# Autodesk Inventor assembly: 20220523_仮機体
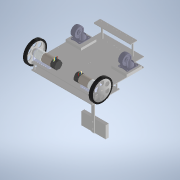
[picture p0: Inventor's stored thumbnail of the model, 180x180]
Saved by Autodesk Inventor 2020 (Build 240168000, 168)
## iProperties
Created: 2022-05-22
Part Number: 20220523_仮機体
Document SubType Name: Assembly
Designer: Naggy
Author: Naggy
## Documents named in this file (15)
- C:\Users\Naggy\Documents\Inventor\robot_design2020\20220523_仮機体.iam
- C:\Users\Naggy\Documents\Inventor\robot_design2020\20220522.ipt
- C:\Users\Naggy\Documents\Inventor\robot_design2020\20220509_知能ロボットキャスタ.ipt
- C:\Users\Naggy\Documents\Inventor\robot_design2020\20220519モータを取り付けるやつ.ipt
- C:\Users\Naggy\Documents\Inventor\robot_design2020\20220519知能ロボットモータとエンコーダ.ipt
- C:\Users\Naggy\Documents\Inventor\robot_design2020\70アルミホイール内径６ (1).ipt
- C:\Users\Naggy\Documents\Inventor\robot_design2020\RD003_キャスタ420G-R32 (3).ipt
- C:\Users\Naggy\Documents\Inventor\robot_design2020\20220508_知能ロボットスペーサ.ipt
- C:\Users\Naggy\Documents\Inventor\robot_design2020\20220523_知能ロボット2階部分.ipt
- C:\Users\Naggy\Documents\Inventor\robot_design2020\20220509_知能ロボットカメラ角棒.ipt
- C:\Users\Naggy\Documents\Inventor\robot_design2020\20220509_知能ロボットカメラ土台.ipt
- C:\Users\Naggy\Documents\Inventor\robot_design2020\20220523_吸引部分吸い.ipt
- C:\Users\Naggy\Documents\Inventor\robot_design2020\20220523_Base Servo v13.iam
- C:\Users\Naggy\Documents\Inventor\robot_design2020\20220523_センサモジュール.ipt
- C:\Users\Naggy\Documents\Inventor\robot_design2020\20220523_スペーサ.ipt
## Components (23 placed, 14 different names)
1. 20220522:1 — メイト:3, メイト:4, メイト:9, メイト:10, メイト:13, メイト:14, メイト:15, メイト:16, メイト:18, メイト:21, メイト:22
2. 20220519モータを取り付けるやつ:2 — メイト:4, メイト:5
3. 20220519モータを取り付けるやつ:3 — メイト:3, メイト:6
4. 20220519知能ロボットモータとエンコーダ:1 — メイト:5, メイト:7
5. 20220519知能ロボットモータとエンコーダ:2 — メイト:6, メイト:8
6. 70アルミホイール内径６ (1):1 — メイト:8
7. 70アルミホイール内径６ (1):2 — メイト:7
8. 20220509_知能ロボットキャスタ:3 — メイト:9, メイト:11
9. RD003_キャスタ420G-R32 (3):3 — メイト:11
10. RD003_キャスタ420G-R32 (3):4 — メイト:12
11. 20220509_知能ロボットキャスタ:4 — メイト:10, メイト:12
12. 20220508_知能ロボットスペーサ:1 — メイト:14
13. 20220508_知能ロボットスペーサ:2 — メイト:16
14. 20220508_知能ロボットスペーサ:3 — メイト:13, メイト:17
15. 20220508_知能ロボットスペーサ:4 — メイト:15
16. 20220523_知能ロボット2階部分:1 — メイト:17
17. 20220509_知能ロボットカメラ角棒:1 — メイト:18, メイト:19
18. 20220509_知能ロボットカメラ土台:1 — メイト:19
19. 20220523_吸引部分吸い:1 — メイト:20
20. 20220523_Base Servo v13:1 [sub-assembly] — メイト:20
21. 20220523_センサモジュール:1 — メイト:23, メイト:24
22. 20220523_スペーサ:1 — メイト:21, メイト:23, メイト:24
23. 20220523_スペーサ:2 — メイト:22
## Relationships (22: Mate 22)
- メイト:3 [Mate]: 20220522:1 ↔ 20220519モータを取り付けるやつ:3
- メイト:4 [Mate]: 20220522:1 ↔ 20220519モータを取り付けるやつ:2
- メイト:5 [Mate]: 20220519モータを取り付けるやつ:2 ↔ 20220519知能ロボットモータとエンコーダ:1
- メイト:6 [Mate]: 20220519モータを取り付けるやつ:3 ↔ 20220519知能ロボットモータとエンコーダ:2
- メイト:7 [Mate]: 20220519知能ロボットモータとエンコーダ:1 ↔ 70アルミホイール内径６ (1):2
- メイト:8 [Mate]: 20220519知能ロボットモータとエンコーダ:2 ↔ 70アルミホイール内径６ (1):1
- メイト:9 [Mate]: 20220522:1 ↔ 20220509_知能ロボットキャスタ:3
- メイト:10 [Mate]: 20220522:1 ↔ 20220509_知能ロボットキャスタ:4
- メイト:11 [Mate]: 20220509_知能ロボットキャスタ:3 ↔ RD003_キャスタ420G-R32 (3):3
- メイト:12 [Mate]: RD003_キャスタ420G-R32 (3):4 ↔ 20220509_知能ロボットキャスタ:4
- メイト:13 [Mate]: 20220522:1 ↔ 20220508_知能ロボットスペーサ:3
- メイト:14 [Mate]: 20220522:1 ↔ 20220508_知能ロボットスペーサ:1
- メイト:15 [Mate]: 20220522:1 ↔ 20220508_知能ロボットスペーサ:4
- メイト:16 [Mate]: 20220522:1 ↔ 20220508_知能ロボットスペーサ:2
- メイト:17 [Mate]: 20220508_知能ロボットスペーサ:3 ↔ 20220523_知能ロボット2階部分:1
- メイト:18 [Mate]: 20220522:1 ↔ 20220509_知能ロボットカメラ角棒:1
- メイト:19 [Mate]: 20220509_知能ロボットカメラ角棒:1 ↔ 20220509_知能ロボットカメラ土台:1
- メイト:20 [Mate]: 20220523_吸引部分吸い:1 ↔ 20220523_Base Servo v13:1
- メイト:21 [Mate]: 20220522:1 ↔ 20220523_スペーサ:1
- メイト:22 [Mate]: 20220522:1 ↔ 20220523_スペーサ:2
- メイト:23 [Mate]: 20220523_センサモジュール:1 ↔ 20220523_スペーサ:1
- メイト:24 [Mate]: 20220523_センサモジュール:1 ↔ 20220523_スペーサ:1
